# Autodesk Inventor assembly: Assembly
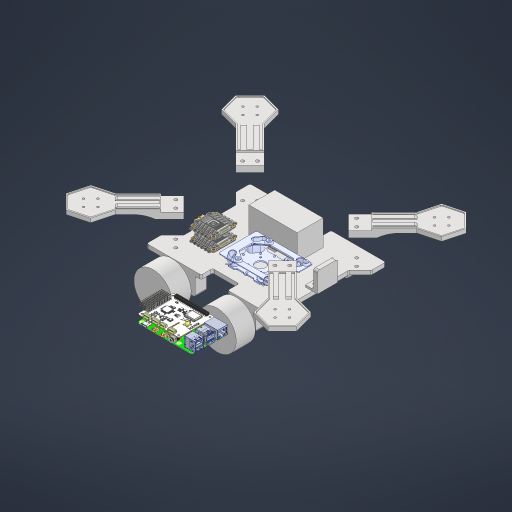
[picture p0: Inventor's stored thumbnail of the model, 512x512]
Saved by Autodesk Inventor 2023 (Build 270158000, 158)
## iProperties
Created: 2023-01-16
Part Number: Assembly
Document SubType Name: Assembly
Designer: Michael
Author: Michael
## Documents named in this file (14)
- \\Mac\Home\Documents\GitHub\SDP-Kepler-1708b\Assembly.iam
- \\Mac\Home\Documents\GitHub\SDP-Kepler-1708b\Base.ipt
- Electronics Panel.ipt
- \\Mac\Home\Documents\GitHub\SDP-Kepler-1708b\navio2\NAVIO2.ipt
- \\Mac\Home\Documents\GitHub\SDP-Kepler-1708b\raspberry-pi-4-model-b\Raspberry Pi 4 Model B.ipt
- \\Mac\Home\Documents\GitHub\SDP-Kepler-1708b\tattu-4s-6750mah-lipo-battery\Tattu_4S_6750mAh_25C\Tattu_4S_6750mAh_25C.ipt
- \\Mac\Home\Documents\GitHub\SDP-Kepler-1708b\LiPo.ipt
- \\Mac\Home\Documents\GitHub\SDP-Kepler-1708b\ESC F45A\F45A.ipt
- \\Mac\Home\Documents\GitHub\SDP-Kepler-1708b\Arm.ipt
- \\Mac\Home\Documents\GitHub\SDP-Kepler-1708b\Top.ipt
- \\Mac\Home\Documents\GitHub\SDP-Kepler-1708b\Camera Mount.ipt
- \\Mac\Home\Documents\GitHub\SDP-Kepler-1708b\Mecanum Wheel.ipt
- \\Mac\Home\Documents\Inventor\VibroNavio2bot_rev_A.ipt
- \\Mac\Home\Documents\GitHub\SDP-Kepler-1708b\navio2\hardware-master\Imported Components\VibroNavio2top_rev_A\VibroNavio2top_rev_A.ipt
## Components (17 placed, 12 different names)
1. Electronics Panel:1 — Mate:25, Mate:26, Mate:33, Mate:34, Mate:35, Mate:36, Flush:5, Mate:39, Mate:40, Mate:41, Mate:42, Mate:43, Mate:44, Mate:45, Mate:47
2. NAVIO2:1 — Mate:5, Flush:1, Flush:2
3. Raspberry Pi 4 Model B:1 — Mate:5, Flush:1, Flush:2, Mate:25
4. Tattu_4S_6750mAh_25C:1 — Mate:40
5. LiPo:1 — Mate:39
6. F45A:1 — Mate:12, Flush:3, Flush:4, Mate:26, Mate:41, Mate:42, Flush:6
7. F45A:2 — Mate:12, Flush:3, Flush:4, Flush:6
8. Arm:2
9. Arm:3
10. Arm:4 — Mate:30, Mate:31, Mate:32
11. Arm:5
12. Top:1 — Mate:30, Mate:31, Mate:32, Mate:33, Flush:5
13. Camera Mount:1 — Mate:34, Mate:35, Mate:36
14. Mecanum Wheel:1 — Mate:43
15. Mecanum Wheel:2 — Mate:44
16. VibroNavio2bot_rev_A:1 — Mate:45, Mate:46, Mate:47
17. VibroNavio2top_rev_A:1 — Mate:46
## Relationships (26: Mate 20, Flush 6)
- Mate:5 (10.16 mm): NAVIO2:1 ↔ Raspberry Pi 4 Model B:1
- Flush:1: NAVIO2:1 ↔ Raspberry Pi 4 Model B:1
- Flush:2: NAVIO2:1 ↔ Raspberry Pi 4 Model B:1
- Mate:12 (12.7 mm): F45A:1 ↔ F45A:2
- Flush:3: F45A:1 ↔ F45A:2
- Flush:4: F45A:1 ↔ F45A:2
- Mate:25: Electronics Panel:1 ↔ Raspberry Pi 4 Model B:1
- Mate:26: Electronics Panel:1 ↔ F45A:1
- Mate:30: Arm:4 ↔ Top:1
- Mate:31: Arm:4 ↔ Top:1
- Mate:32: Arm:4 ↔ Top:1
- Mate:33 (44.45 mm): Electronics Panel:1 ↔ Top:1
- Mate:34: Electronics Panel:1 ↔ Camera Mount:1
- Mate:35: Electronics Panel:1 ↔ Camera Mount:1
- Mate:36: Electronics Panel:1 ↔ Camera Mount:1
- Flush:5: Electronics Panel:1 ↔ Top:1
- Mate:39: Electronics Panel:1 ↔ LiPo:1
- Mate:40: Electronics Panel:1 ↔ Tattu_4S_6750mAh_25C:1
- Mate:41: Electronics Panel:1 ↔ F45A:1
- Mate:42: Electronics Panel:1 ↔ F45A:1
- Flush:6: F45A:1 ↔ F45A:2
- Mate:43 (12.7 mm): Electronics Panel:1 ↔ Mecanum Wheel:1
- Mate:44 (12.7 mm): Electronics Panel:1 ↔ Mecanum Wheel:2
- Mate:45: Electronics Panel:1 ↔ VibroNavio2bot_rev_A:1
- Mate:46: VibroNavio2bot_rev_A:1 ↔ VibroNavio2top_rev_A:1
- Mate:47: Electronics Panel:1 ↔ VibroNavio2bot_rev_A:1
